# Autodesk Inventor assembly: s-assy-frame_bolt
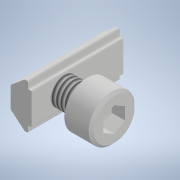
[picture p0: Inventor's stored thumbnail of the model, 180x180]
Saved by Autodesk Inventor 2022 (Build 260153000, 153)
## iProperties
Created: 2021-09-21
Part Number: s-assy-frame_bolt
Document SubType Name: Assembly
Designer: yuto6
Author: yuto6
## Documents named in this file (3)
- C:\Users\yuto6\Box\Public_Share\キャチロボバトルコンテスト2021\CAD\catchrobo_hardware\assy-shooter\s-assy-frame_bolt.iam
- C:\Users\yuto6\Box\Public_Share\キャチロボバトルコンテスト2021\CAD\catchrobo_hardware\assy-shooter\HNTP5-5.ipt
- C:\Users\yuto6\Box\Public_Share\キャチロボバトルコンテスト2021\CAD\catchrobo_hardware\assy-shooter\CB5-8.ipt
## Components (2 placed, 2 different names)
1. HNTP5-5:1 — メイト:1, メイト:2
2. CB5-8:1 — メイト:1, メイト:2
## Relationships (2: Mate 2)
- メイト:1 [Mate]: HNTP5-5:1 ↔ CB5-8:1
- メイト:2 [Mate] (4.3 mm): HNTP5-5:1 ↔ CB5-8:1
